# Autodesk Inventor assembly: YAxis_Carriage
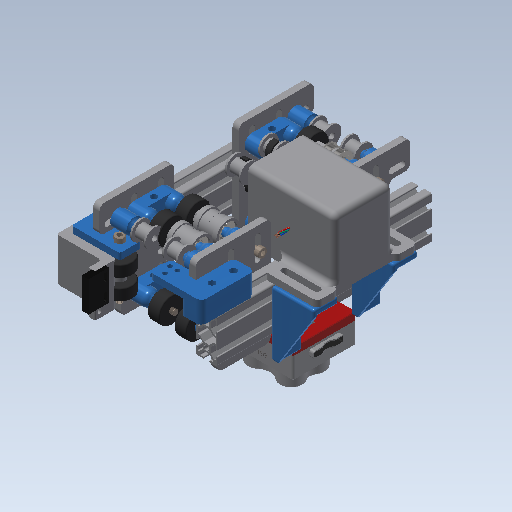
[picture p0: Inventor's stored thumbnail of the model, 512x512]
Saved by Autodesk Inventor 2021 (Build 250183000, 183)
## iProperties
Created: 2021-02-02
Part Number: YAxis_Carriage
Document SubType Name: Assembly
Designer: Jorian Brusind
Author: Jorian Brusind
## Documents named in this file (23)
- C:\Users\Jorian Brusind\Documents\GitHub\PersonalProjects\HyperRail\Inventor Files\YAxis_Carriage.iam
- C:\Users\Jorian Brusind\Documents\GitHub\PersonalProjects\HyperRail\Inventor Files\SmallBelt_Pulley.ipt
- C:\Users\Jorian Brusind\Documents\GitHub\PersonalProjects\Inventor Projects\Useful models\Metric bolt\Bolt M3 30mm.ipt
- C:\Users\Jorian Brusind\Documents\GitHub\PersonalProjects\HyperRail\Inventor Files\small_belt_loop.ipt
- C:\Users\Jorian Brusind\Documents\GitHub\PersonalProjects\HyperRail\PCB Files\Integrated Stepper Motor Driver\ExportSTEP\Main.iam
- C:\Users\Jorian Brusind\Documents\GitHub\PersonalProjects\HyperRail\Inventor Files\rededge-micasense-1.snapshot.3\PND_CAM_MSRE.ipt
- C:\Users\Jorian Brusind\Documents\GitHub\PersonalProjects\HyperRail\Inventor Files\NEMA17_Shroud.ipt
- C:\Users\Jorian Brusind\Documents\GitHub\PersonalProjects\HyperRail\Inventor Files\Buffer.iam
- C:\Users\Jorian Brusind\Documents\GitHub\PersonalProjects\HyperRail\Inventor Files\X_Carriage_V2_0.iam
- C:\Users\Jorian Brusind\Documents\GitHub\PersonalProjects\HyperRail\Inventor Files\X_CarriageR_V2_0.iam
- C:\Users\Jorian Brusind\Documents\GitHub\PersonalProjects\HyperRail\Inventor Files\X_CarriageR_V2_1.iam
- C:\Users\Jorian Brusind\Documents\GitHub\PersonalProjects\HyperRail\Inventor Files\X_Carriage_V2_1.iam
- C:\Users\Jorian Brusind\Documents\GitHub\PersonalProjects\Inventor Projects\Useful models\8020_Sets\IPT_20_Series\IPT_20_Series\20-2040_200mm.ipt
- C:\Users\Jorian Brusind\Documents\GitHub\PersonalProjects\HyperRail\Inventor Files\10mm_Idle_Pulley_3M.ipt
- C:\Users\Jorian Brusind\Documents\GitHub\PersonalProjects\HyperRail\Inventor Files\McMaster Files\Hex Standoffs\95947A725_Aluminum Female Threaded Hex Standoff.ipt
- C:\Users\Jorian Brusind\Documents\GitHub\PersonalProjects\Inventor Projects\Useful models\Metric bolt\Bolt M5 45mm.ipt
- C:\Users\Jorian Brusind\Documents\GitHub\PersonalProjects\HyperRail\Inventor Files\nema17-x-40-1.snapshot.7\NEMA17 x 40.ipt
- C:\Users\Jorian Brusind\Documents\GitHub\PersonalProjects\HyperRail\Inventor Files\RightAngle_Bracket.ipt
- C:\Users\Jorian Brusind\Documents\GitHub\PersonalProjects\HyperRail\Inventor Files\59145_Actuator.ipt
- C:\Users\Jorian Brusind\Documents\GitHub\PersonalProjects\HyperRail\Inventor Files\MagnetHolder.ipt
- C:\Users\Jorian Brusind\Documents\GitHub\PersonalProjects\HyperRail\Inventor Files\CableChain_Mount.ipt
- C:\Users\Jorian Brusind\Documents\GitHub\PersonalProjects\HyperRail\Inventor Files\Buffer_L.iam
- C:\Users\Jorian Brusind\Documents\GitHub\PersonalProjects\HyperRail\Inventor Files\MagnetActuatorHolder.ipt
## Components (43 placed, 22 different names)
1. SmallBelt_Pulley:1 — Mate:37, Flush:94, Mate:208, Flush:102, Mate:238
2. small_belt_loop:1 — Mate:37, Mate:213, Angle:1
3. Main:1 [sub-assembly] — Mate:209, Mate:210, Mate:211
4. PND_CAM_MSRE:1 — Mate:188, Flush:95, Mate:189
5. 20-2040_200mm:1 — Flush:74, Flush:75, Mate:151, Mate:157, Flush:76, Flush:77, Mate:161, Flush:80, Mate:175, Flush:89, Mate:188, Mate:243, Mate:250, Flush:107, Flush:108, Flush:113, Mate:255, Flush:114, Mate:259, Flush:116, Mate:263
6. 20-2040_200mm:2 — Flush:74, Flush:75, Mate:155, Mate:156, Mate:160, Mate:174, Flush:95, Mate:223, Mate:224, Mate:227, Flush:112, Mate:253, Mate:254
7. X_CarriageR_V2_0:4 [sub-assembly] — Mate:161, Flush:80, Mate:162, Flush:85, Mate:167, Flush:86, Flush:90, Mate:186, Mate:200, Mate:201, Mate:202, Mate:233, Flush:106, Mate:268, Mate:269, Mate:270
8. X_Carriage_V2_1:3 [sub-assembly] — Mate:160, Flush:85, Mate:167, Mate:186, Mate:198, Mate:199, Mate:205, Mate:237, Mate:238, Mate:275, Mate:276, Mate:277
9. Buffer:4 [sub-assembly] — Mate:157, Flush:76, Flush:77, Mate:162
10. Bolt M3 30mm:2 — Mate:183, Mate:184, Mate:219
11. X_Carriage_V2_0:1 [sub-assembly] — Mate:175, Flush:86, Flush:87, Flush:88, Flush:89, Flush:90, Mate:177, Mate:187, Mate:206, Mate:207, Flush:106, Mate:235, Mate:266, Mate:267, Mate:271
12. X_CarriageR_V2_1:1 [sub-assembly] — Mate:174, Flush:87, Flush:88, Mate:177, Mate:187, Mate:189, Mate:203, Mate:204, Mate:217, Mate:234, Mate:236, Mate:272, Mate:273, Mate:274
13. 10mm_Idle_Pulley_3M:2 — Flush:91, Mate:220
14. 10mm_Idle_Pulley_3M:4 — Flush:91, Flush:94, Mate:183, Mate:184
15. 95947A725_Aluminum Female Threaded Hex Standoff:2 — Mate:232, Mate:233, Mate:237
16. 95947A725_Aluminum Female Threaded Hex Standoff:3 — Mate:228, Mate:230, Mate:236
17. 95947A725_Aluminum Female Threaded Hex Standoff:4 — Mate:229, Mate:234, Mate:235
18. Bolt M5 45mm:1 — Mate:201, Flush:96, Mate:202, Flush:101, Mate:232
19. Bolt M5 45mm:2 — Mate:198, Flush:97
20. Bolt M5 45mm:3 — Mate:207, Flush:100, Flush:101, Mate:228
21. Bolt M5 45mm:4 — Mate:206, Flush:100, Mate:229
22. Bolt M5 45mm:5 — Mate:200, Flush:96
23. Bolt M5 45mm:6 — Mate:203, Flush:98, Flush:99, Mate:230
24. Bolt M5 45mm:7 — Mate:204, Flush:98
25. Bolt M5 45mm:8 — Mate:199, Flush:97, Flush:99, Mate:205
26. NEMA17 x 40:1 — Mate:208, Mate:209, Mate:210, Mate:211, Mate:213, Flush:102, Mate:214, Mate:215, Mate:216
27. NEMA17_Shroud:1 — Mate:214, Mate:215, Mate:216, Mate:217, Mate:219, Mate:220, Mate:225, Mate:226, Flush:104, Flush:105, Mate:227, Angle:1
28. RightAngle_Bracket:1 — Mate:224, Mate:226, Flush:104
29. RightAngle_Bracket:2 — Mate:223, Mate:225, Flush:105
30. 59145_Actuator:3 — Mate:247, Angle:4
31. MagnetHolder:2 — Mate:243, Mate:247, Angle:4, Mate:250, Flush:107, Flush:108
32. CableChain_Mount:1 — Flush:112, Mate:253, Mate:254
33. Buffer_L:1 [sub-assembly] — Flush:113, Mate:255, Flush:114
34. 59145_Actuator:5 — Mate:264, Flush:117, Mate:265
35. MagnetActuatorHolder:1 — Mate:259, Flush:116, Mate:263, Mate:264, Flush:117, Mate:265
36. Bolt M5 45mm:9 — Mate:267
37. Bolt M5 45mm:10 — Mate:266, Mate:271
38. Bolt M5 45mm:11 — Mate:269, Mate:270
39. Bolt M5 45mm:12 — Mate:268
40. Bolt M5 45mm:13 — Mate:273
41. Bolt M5 45mm:14 — Mate:272, Mate:274
42. Bolt M5 45mm:17 — Mate:275, Mate:277
43. Bolt M5 45mm:18 — Mate:276
## Relationships (114: Mate 77, Flush 35, Angle 2)
- Mate:37 (2 mm): SmallBelt_Pulley:1 ↔ small_belt_loop:1
- Flush:74: 20-2040_200mm:1 ↔ 20-2040_200mm:2
- Flush:75: 20-2040_200mm:1 ↔ 20-2040_200mm:2
- Mate:151: 20-2040_200mm:1
- Mate:155: 20-2040_200mm:2
- Mate:156: 20-2040_200mm:2
- Mate:157: 20-2040_200mm:1 ↔ Buffer:4
- Flush:76: 20-2040_200mm:1 ↔ Buffer:4
- Flush:77: 20-2040_200mm:1 ↔ Buffer:4
- Mate:160: 20-2040_200mm:2 ↔ X_Carriage_V2_1:3
- Mate:161: 20-2040_200mm:1 ↔ X_CarriageR_V2_0:4
- Flush:80: 20-2040_200mm:1 ↔ X_CarriageR_V2_0:4
- Mate:162 (4 mm): X_CarriageR_V2_0:4 ↔ Buffer:4
- Flush:85: X_CarriageR_V2_0:4 ↔ X_Carriage_V2_1:3
- Mate:167: X_CarriageR_V2_0:4 ↔ X_Carriage_V2_1:3
- Mate:174: 20-2040_200mm:2 ↔ X_CarriageR_V2_1:1
- Mate:175: 20-2040_200mm:1 ↔ X_Carriage_V2_0:1
- Flush:86: X_CarriageR_V2_0:4 ↔ X_Carriage_V2_0:1
- Flush:87: X_Carriage_V2_0:1 ↔ X_CarriageR_V2_1:1
- Flush:88: X_Carriage_V2_0:1 ↔ X_CarriageR_V2_1:1
- Flush:89: 20-2040_200mm:1 ↔ X_Carriage_V2_0:1
- Flush:90: X_CarriageR_V2_0:4 ↔ X_Carriage_V2_0:1
- Mate:177: X_Carriage_V2_0:1 ↔ X_CarriageR_V2_1:1
- Flush:91: 10mm_Idle_Pulley_3M:2 ↔ 10mm_Idle_Pulley_3M:4
- Flush:94: SmallBelt_Pulley:1 ↔ 10mm_Idle_Pulley_3M:4
- Mate:183: Bolt M3 30mm:2 ↔ 10mm_Idle_Pulley_3M:4
- Mate:184: Bolt M3 30mm:2 ↔ 10mm_Idle_Pulley_3M:4
- Mate:186: X_CarriageR_V2_0:4 ↔ X_Carriage_V2_1:3
- Mate:187: X_Carriage_V2_0:1 ↔ X_CarriageR_V2_1:1
- Mate:188 (20 mm): PND_CAM_MSRE:1 ↔ 20-2040_200mm:1
- Flush:95: PND_CAM_MSRE:1 ↔ 20-2040_200mm:2
- Mate:189 (0.5 mm): PND_CAM_MSRE:1 ↔ X_CarriageR_V2_1:1
- Mate:198: X_Carriage_V2_1:3 ↔ Bolt M5 45mm:2
- Mate:199: X_Carriage_V2_1:3 ↔ Bolt M5 45mm:8
- Mate:200: X_CarriageR_V2_0:4 ↔ Bolt M5 45mm:5
- Mate:201: X_CarriageR_V2_0:4 ↔ Bolt M5 45mm:1
- Flush:96: Bolt M5 45mm:1 ↔ Bolt M5 45mm:5
- Mate:202: X_CarriageR_V2_0:4 ↔ Bolt M5 45mm:1
- Flush:97: Bolt M5 45mm:2 ↔ Bolt M5 45mm:8
- Mate:203: X_CarriageR_V2_1:1 ↔ Bolt M5 45mm:6
- Mate:204: X_CarriageR_V2_1:1 ↔ Bolt M5 45mm:7
- Flush:98: Bolt M5 45mm:6 ↔ Bolt M5 45mm:7
- Flush:99: Bolt M5 45mm:6 ↔ Bolt M5 45mm:8
- Mate:205: X_Carriage_V2_1:3 ↔ Bolt M5 45mm:8
- Mate:206: X_Carriage_V2_0:1 ↔ Bolt M5 45mm:4
- Mate:207: X_Carriage_V2_0:1 ↔ Bolt M5 45mm:3
- Flush:100: Bolt M5 45mm:3 ↔ Bolt M5 45mm:4
- Flush:101: Bolt M5 45mm:1 ↔ Bolt M5 45mm:3
- Mate:208: SmallBelt_Pulley:1 ↔ NEMA17 x 40:1
- Mate:209: Main:1 ↔ NEMA17 x 40:1
- Mate:210: Main:1 ↔ NEMA17 x 40:1
- Mate:211 (8 mm): Main:1 ↔ NEMA17 x 40:1
- Mate:213: small_belt_loop:1 ↔ NEMA17 x 40:1
- Flush:102: SmallBelt_Pulley:1 ↔ NEMA17 x 40:1
- Mate:214: NEMA17 x 40:1 ↔ NEMA17_Shroud:1
- Mate:215: NEMA17 x 40:1 ↔ NEMA17_Shroud:1
- Mate:216: NEMA17 x 40:1 ↔ NEMA17_Shroud:1
- Mate:217 (3 mm): X_CarriageR_V2_1:1 ↔ NEMA17_Shroud:1
- Mate:219: Bolt M3 30mm:2 ↔ NEMA17_Shroud:1
- Mate:220: 10mm_Idle_Pulley_3M:2 ↔ NEMA17_Shroud:1
- Mate:223: 20-2040_200mm:2 ↔ RightAngle_Bracket:2
- Mate:224: 20-2040_200mm:2 ↔ RightAngle_Bracket:1
- Mate:225: NEMA17_Shroud:1 ↔ RightAngle_Bracket:2
- Mate:226: NEMA17_Shroud:1 ↔ RightAngle_Bracket:1
- Flush:104: NEMA17_Shroud:1 ↔ RightAngle_Bracket:1
- Flush:105: NEMA17_Shroud:1 ↔ RightAngle_Bracket:2
- Mate:227: 20-2040_200mm:2 ↔ NEMA17_Shroud:1
- Mate:228: 95947A725_Aluminum Female Threaded Hex Standoff:3 ↔ Bolt M5 45mm:3
- Mate:229: 95947A725_Aluminum Female Threaded Hex Standoff:4 ↔ Bolt M5 45mm:4
- Mate:230: 95947A725_Aluminum Female Threaded Hex Standoff:3 ↔ Bolt M5 45mm:6
- Mate:232: 95947A725_Aluminum Female Threaded Hex Standoff:2 ↔ Bolt M5 45mm:1
- Mate:233: X_CarriageR_V2_0:4 ↔ 95947A725_Aluminum Female Threaded Hex Standoff:2
- Flush:106: X_CarriageR_V2_0:4 ↔ X_Carriage_V2_0:1
- Mate:234: X_CarriageR_V2_1:1 ↔ 95947A725_Aluminum Female Threaded Hex Standoff:4
- Mate:235: X_Carriage_V2_0:1 ↔ 95947A725_Aluminum Female Threaded Hex Standoff:4
- Mate:236: X_CarriageR_V2_1:1 ↔ 95947A725_Aluminum Female Threaded Hex Standoff:3
- Mate:237: X_Carriage_V2_1:3 ↔ 95947A725_Aluminum Female Threaded Hex Standoff:2
- Angle:1 (0 deg): small_belt_loop:1 ↔ NEMA17_Shroud:1
- Mate:238: SmallBelt_Pulley:1 ↔ X_Carriage_V2_1:3
- [Mate]: 59145_Actuator:3 ↔ MagnetHolder:2
- Mate:243: 20-2040_200mm:1 ↔ MagnetHolder:2
- Mate:247: 59145_Actuator:3 ↔ MagnetHolder:2
- Angle:4 (0 deg): 59145_Actuator:3 ↔ MagnetHolder:2
- Mate:250: 20-2040_200mm:1 ↔ MagnetHolder:2
- Flush:107: 20-2040_200mm:1 ↔ MagnetHolder:2
- Flush:108: 20-2040_200mm:1 ↔ MagnetHolder:2
- Flush:112: 20-2040_200mm:2 ↔ CableChain_Mount:1
- Mate:253 (-5 mm): 20-2040_200mm:2 ↔ CableChain_Mount:1
- Mate:254: 20-2040_200mm:2 ↔ CableChain_Mount:1
- Flush:113: 20-2040_200mm:1 ↔ Buffer_L:1
- Mate:255: 20-2040_200mm:1 ↔ Buffer_L:1
- Flush:114: 20-2040_200mm:1 ↔ Buffer_L:1
- Mate:259: 20-2040_200mm:1 ↔ MagnetActuatorHolder:1
- Flush:116: 20-2040_200mm:1 ↔ MagnetActuatorHolder:1
- Mate:263: 20-2040_200mm:1 ↔ MagnetActuatorHolder:1
- Mate:264: 59145_Actuator:5 ↔ MagnetActuatorHolder:1
- Flush:117: 59145_Actuator:5 ↔ MagnetActuatorHolder:1
- Mate:265: 59145_Actuator:5 ↔ MagnetActuatorHolder:1
- [Flush]: Bolt M5 45mm:9 ↔ Bolt M5 45mm:10
- [Flush]: Bolt M5 45mm:11 ↔ Bolt M5 45mm:12
- Mate:266: X_Carriage_V2_0:1 ↔ Bolt M5 45mm:10
- Mate:267: X_Carriage_V2_0:1 ↔ Bolt M5 45mm:9
- Mate:268: X_CarriageR_V2_0:4 ↔ Bolt M5 45mm:12
- Mate:269: X_CarriageR_V2_0:4 ↔ Bolt M5 45mm:11
- Mate:270: X_CarriageR_V2_0:4 ↔ Bolt M5 45mm:11
- Mate:271: X_Carriage_V2_0:1 ↔ Bolt M5 45mm:10
- [Flush]: Bolt M5 45mm:13 ↔ Bolt M5 45mm:14
- Mate:272: X_CarriageR_V2_1:1 ↔ Bolt M5 45mm:14
- Mate:273: X_CarriageR_V2_1:1 ↔ Bolt M5 45mm:13
- Mate:274: X_CarriageR_V2_1:1 ↔ Bolt M5 45mm:14
- [Flush]: Bolt M5 45mm:17 ↔ Bolt M5 45mm:18
- Mate:275: X_Carriage_V2_1:3 ↔ Bolt M5 45mm:17
- Mate:276: X_Carriage_V2_1:3 ↔ Bolt M5 45mm:18
- Mate:277: X_Carriage_V2_1:3 ↔ Bolt M5 45mm:17
## Named parameters: d431_d430 = 0 mm, d498_d374 = 0 mm, d499_d374 = 0 mm, d506_d498_d374 = 0 mm, d511_d506_d498_d374 = 0 mm
